# Autodesk Inventor assembly: Full Wheel
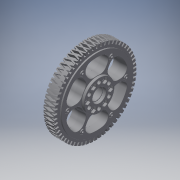
[picture p0: Inventor's stored thumbnail of the model, 180x180]
Saved by Autodesk Inventor 2019 (Build 230136000, 136)
## iProperties
Company: Unknown
Created: 2008-07-13
Part Number: Full Wheel
Description: Unknown
Document SubType Name: Assembly
Designer: lopez.xavier
Sending System: Unknown
Preprocessor: XStep 1.0
Title: F:/6Plaction_asm.stp
Author: Unknown
Revision Number: NONE
## Documents named in this file (4)
- \\fs1\studentusers\class22\Rachala.Rohit\documents\Laptop Inventor\2019Robot\Full Wheel.iam
- \\fs1\studentusers\class22\Rachala.Rohit\documents\Laptop Inventor\2019Robot\6MW_d01.ipt
- \\fs1\studentusers\class22\Rachala.Rohit\documents\Laptop Inventor\2019Robot\10-32_locknut.ipt
- \\fs1\studentusers\class22\Rachala.Rohit\documents\Laptop Inventor\2019Robot\Tread.ipt
## Components (9 placed, 3 different names)
1. 6MW_d01 — Mate:1
2. 6MW_d01:1 — Flush:1
3. 10-32_locknut
4. 10-32_locknut:1
5. 10-32_locknut:2
6. 10-32_locknut:3
7. 10-32_locknut:4
8. 10-32_locknut:5
9. Tread:1 — Mate:1, Flush:1
## Relationships (2: Mate 1, Flush 1)
- Mate:1: 6MW_d01 ↔ Tread:1
- Flush:1 (3.048 mm): 6MW_d01:1 ↔ Tread:1
